# Autodesk Inventor assembly: Hand
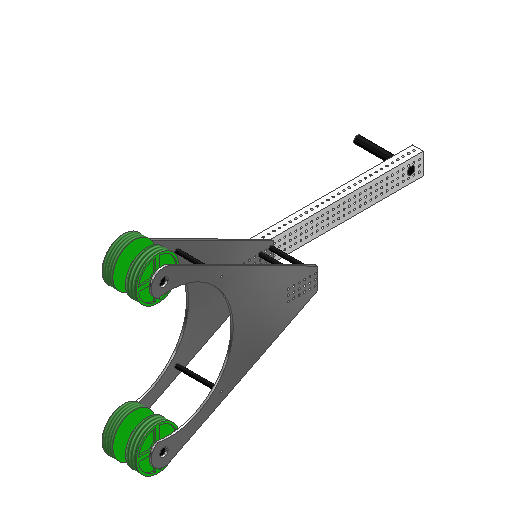
[picture p0: Inventor's stored thumbnail of the model, 512x512]
Saved by Autodesk Inventor 2025.3 (Build 293356000, 356)
## iProperties
Created: 2026-05-13
Part Number: Hand
Document SubType Name: Assembly
Designer: djair.oliveira
Author: djair.oliveira
## Documents named in this file (7)
- C:\Users\djair.oliveira\Documents\GitHub\MT_2026\CAD\Model B\Hand\Hand.iam
- C:\Users\djair.oliveira\Documents\GitHub\MT_2026\CAD\Model B\Hand\Forja - Base1 Hand.ipt
- C:\Users\djair.oliveira\Documents\GitHub\MT_2026\CAD\Model B\Hand\Articulation Hand.ipt
- C:\Users\djair.oliveira\Documents\GitHub\MT_2026\CAD\Model B\Hand\Chapa Base - Hand.ipt
- C:\Users\djair.oliveira\Documents\GitHub\MT_2026\CAD\Model B\Hand\Coletor - Hand.ipt
- C:\Users\djair.oliveira\Documents\GitHub\MT_2026\CAD\Model B\Hand\Suporte - Chapa Base Hand.ipt
- C:\Users\djair.oliveira\Documents\GitHub\MT_2026\CAD\Model B\Hand\Suporte - Chapa Base Hand_MIR.ipt
## Components (12 placed, 6 different names)
1. Forja - Base1 Hand:1 — Alinhado:1, Coincidente:1, Coincidente:2, Coincidente:3, Coincidente:4, Alinhado:2
2. Articulation Hand:1 — Alinhado:1, Coincidente:1
3. Chapa Base - Hand:1 — Coincidente:2, Coincidente:3, Coincidente:4, Coincidente:5, Coincidente:6, Coincidente:7, Coincidente:8, Coincidente:12, Coincidente:13, Coincidente:14, Coincidente:15, Coincidente:16, Coincidente:18, Coincidente:19, Coincidente:20, Coincidente:21, Coincidente:22
4. Chapa Base - Hand:2 — Coincidente:9, Coincidente:10, Coincidente:11
5. Coletor - Hand:1 — Coincidente:5, Coincidente:6, Coincidente:10
6. Coletor - Hand:2 — Coincidente:7, Coincidente:8, Coincidente:9, Coincidente:11
7. Suporte - Chapa Base Hand:1 — Coincidente:13, Coincidente:21
8. Suporte - Chapa Base Hand:2 — Coincidente:15, Coincidente:18
9. Suporte - Chapa Base Hand:3 — Coincidente:16, Coincidente:22
10. Suporte - Chapa Base Hand:5 — Coincidente:14, Coincidente:20
11. Suporte - Chapa Base Hand:6 — Coincidente:12, Coincidente:19
12. Suporte - Chapa Base Hand_MIR:1
## Relationships (23: Mate 21, Flush 2)
- Alinhado:1 [Flush]: Forja - Base1 Hand:1 ↔ Articulation Hand:1
- Coincidente:1 [Mate]: Forja - Base1 Hand:1 ↔ Articulation Hand:1
- Coincidente:2 [Mate]: Forja - Base1 Hand:1 ↔ Chapa Base - Hand:1
- Coincidente:3 [Mate]: Forja - Base1 Hand:1 ↔ Chapa Base - Hand:1
- Coincidente:4 [Mate]: Forja - Base1 Hand:1 ↔ Chapa Base - Hand:1
- Coincidente:5 [Mate]: Chapa Base - Hand:1 ↔ Coletor - Hand:1
- Coincidente:6 [Mate]: Chapa Base - Hand:1 ↔ Coletor - Hand:1
- Coincidente:7 [Mate]: Chapa Base - Hand:1 ↔ Coletor - Hand:2
- Coincidente:8 [Mate]: Chapa Base - Hand:1 ↔ Coletor - Hand:2
- Coincidente:9 [Mate]: Chapa Base - Hand:2 ↔ Coletor - Hand:2
- Coincidente:10 [Mate]: Chapa Base - Hand:2 ↔ Coletor - Hand:1
- Coincidente:11 [Mate]: Chapa Base - Hand:2 ↔ Coletor - Hand:2
- Coincidente:12 [Mate]: Chapa Base - Hand:1 ↔ Suporte - Chapa Base Hand:6
- Coincidente:13 [Mate]: Chapa Base - Hand:1 ↔ Suporte - Chapa Base Hand:1
- Coincidente:14 [Mate]: Chapa Base - Hand:1 ↔ Suporte - Chapa Base Hand:5
- Coincidente:15 [Mate]: Chapa Base - Hand:1 ↔ Suporte - Chapa Base Hand:2
- Coincidente:16 [Mate]: Chapa Base - Hand:1 ↔ Suporte - Chapa Base Hand:3
- Coincidente:18 [Mate]: Chapa Base - Hand:1 ↔ Suporte - Chapa Base Hand:2
- Coincidente:19 [Mate]: Chapa Base - Hand:1 ↔ Suporte - Chapa Base Hand:6
- Coincidente:20 [Mate]: Chapa Base - Hand:1 ↔ Suporte - Chapa Base Hand:5
- Coincidente:21 [Mate]: Chapa Base - Hand:1 ↔ Suporte - Chapa Base Hand:1
- Alinhado:2 [Flush] (-25.4 mm): Forja - Base1 Hand:1
- Coincidente:22 [Mate]: Chapa Base - Hand:1 ↔ Suporte - Chapa Base Hand:3
